# Autodesk Inventor assembly: BOX_PART
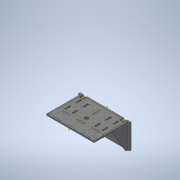
[picture p0: Inventor's stored thumbnail of the model, 180x180]
Saved by Autodesk Inventor 2020 (Build 240168000, 168)
## iProperties
Created: 2019-12-17
Part Number: BOX_PART
Document SubType Name: Assembly
Designer: fabfarm
Author: fabfarm
## Documents named in this file (9)
- D:\fablab\sawbench\BOX_PART.iam
- D:\fablab\sawbench\Side_one.ipt
- D:\fablab\sawbench\Side_two.ipt
- D:\fablab\sawbench\TableSaw_Bench3.ipt
- D:\fablab\sawbench\bottom-case.ipt
- D:\fablab\sawbench\open_case.ipt
- D:\fablab\sawbench\bottom-tool_part.ipt
- D:\fablab\sawbench\top_part.ipt
- D:\fablab\sawbench\Bracket.ipt
## Components (10 placed, 8 different names)
1. Side_one:1 — Flush:4, Flush:5, Symmetry:1, Placage:11, Placage:17, Placage:26, Placage:33
2. Side_two:1 — Mate:10, Flush:4, Flush:7, Symmetry:2, Affleurement:12, Affleurement:16, Placage:25
3. TableSaw_Bench3:1 — Affleurement:13, Placage:15, Affleurement:14, Placage:20, Placage:22, Placage:23
4. Side_one:2 — Flush:7, Flush:10, Symmetry:1, Affleurement:11, Affleurement:12, Placage:14, Placage:16, Affleurement:17, Placage:24, Placage:25, Placage:34, Placage:35
5. bottom-case:1 — Mate:10, Flush:5, Placage:11, Affleurement:11, Placage:16, Placage:20
6. open_case:1 — Flush:10, Symmetry:2, Placage:14, Placage:21, Placage:24
7. bottom-tool_part:1 — Placage:17, Affleurement:16, Affleurement:17
8. top_part:1 — Placage:21, Placage:22, Placage:23, Placage:27, Placage:31
9. Bracket:1 — Placage:26, Placage:27, Placage:33
10. Bracket:4 — Placage:31, Placage:34, Placage:35
## Relationships (30: Mate 18, Flush 10, Symmetry 2)
- Mate:10: Side_two:1 ↔ bottom-case:1
- Flush:4: Side_one:1 ↔ Side_two:1
- Flush:5: Side_one:1 ↔ bottom-case:1
- Flush:7: Side_two:1 ↔ Side_one:2
- Flush:10: Side_one:2 ↔ open_case:1
- Symmetry:1: Side_one:1 ↔ Side_one:2
- Symmetry:2: Side_two:1 ↔ open_case:1
- Placage:11 [Mate]: Side_one:1 ↔ bottom-case:1
- Affleurement:11 [Flush]: Side_one:2 ↔ bottom-case:1
- Affleurement:12 [Flush]: Side_two:1 ↔ Side_one:2
- Placage:14 [Mate]: Side_one:2 ↔ open_case:1
- Affleurement:13 [Flush]: TableSaw_Bench3:1
- Placage:15 [Mate]: TableSaw_Bench3:1
- Affleurement:14 [Flush]: TableSaw_Bench3:1
- Placage:16 [Mate]: Side_one:2 ↔ bottom-case:1
- Placage:17 [Mate]: Side_one:1 ↔ bottom-tool_part:1
- Affleurement:16 [Flush]: Side_two:1 ↔ bottom-tool_part:1
- Affleurement:17 [Flush]: Side_one:2 ↔ bottom-tool_part:1
- Placage:20 [Mate]: TableSaw_Bench3:1 ↔ bottom-case:1
- Placage:21 [Mate]: open_case:1 ↔ top_part:1
- Placage:22 [Mate]: TableSaw_Bench3:1 ↔ top_part:1
- Placage:23 [Mate]: TableSaw_Bench3:1 ↔ top_part:1
- Placage:24 [Mate]: Side_one:2 ↔ open_case:1
- Placage:25 [Mate]: Side_two:1 ↔ Side_one:2
- Placage:26 [Mate]: Side_one:1 ↔ Bracket:1
- Placage:27 [Mate]: top_part:1 ↔ Bracket:1
- Placage:31 [Mate]: top_part:1 ↔ Bracket:4
- Placage:33 [Mate]: Side_one:1 ↔ Bracket:1
- Placage:34 [Mate]: Side_one:2 ↔ Bracket:4
- Placage:35 [Mate]: Side_one:2 ↔ Bracket:4
